# Autodesk Inventor assembly: mirrorHolder
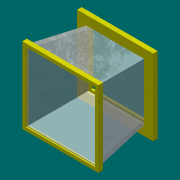
[picture p0: Inventor's stored thumbnail of the model, 180x180]
Saved by Autodesk Inventor 2016 (Build 200138000, 138)
## iProperties
Created: 2015-10-27
Part Number: mirrorHolder
Document SubType Name: Assembly
Designer: Sawaiz
Author: Sawaiz
## Documents named in this file (5)
- C:\Users\Sawaiz\OneDrive\projects\modularRICH\mirror\mirrorHolder.iam
- C:\Users\Sawaiz\OneDrive\projects\modularRICH\mirror\mirrorFrontFrame.ipt
- C:\Users\Sawaiz\OneDrive\projects\modularRICH\mirror\mirrorSides.ipt
- C:\Users\Sawaiz\OneDrive\projects\modularRICH\mirror\mirrorTopBottom.ipt
- C:\Users\Sawaiz\OneDrive\projects\modularRICH\mirror\mirrorBackFrame.ipt
## Components (6 placed, 4 different names)
1. mirrorFrontFrame:1 — Mate:7, Mate:8, Mate:9
2. mirrorSides:1 — Flush:2, Mate:5, Mate:6, Mate:9
3. mirrorTopBottom:1 — Flush:1, Mate:3, Mate:4, Mate:5, Mate:6
4. mirrorSides:2 — Flush:3, Mate:1, Mate:2, Mate:3, Mate:4
5. mirrorTopBottom:2 — Flush:1, Flush:2, Flush:3, Mate:1, Mate:2, Mate:7, Mate:8, Flush:4
6. mirrorBackFrame:1 — Flush:4
## Relationships (13: Mate 9, Flush 4)
- Flush:1: mirrorTopBottom:1 ↔ mirrorTopBottom:2
- Flush:2: mirrorSides:1 ↔ mirrorTopBottom:2
- Flush:3: mirrorSides:2 ↔ mirrorTopBottom:2
- Mate:1: mirrorSides:2 ↔ mirrorTopBottom:2
- Mate:2: mirrorSides:2 ↔ mirrorTopBottom:2
- Mate:3: mirrorTopBottom:1 ↔ mirrorSides:2
- Mate:4: mirrorTopBottom:1 ↔ mirrorSides:2
- Mate:5: mirrorSides:1 ↔ mirrorTopBottom:1
- Mate:6: mirrorSides:1 ↔ mirrorTopBottom:1
- Mate:7: mirrorFrontFrame:1 ↔ mirrorTopBottom:2
- Mate:8: mirrorFrontFrame:1 ↔ mirrorTopBottom:2
- Mate:9: mirrorFrontFrame:1 ↔ mirrorSides:1
- Flush:4: mirrorTopBottom:2 ↔ mirrorBackFrame:1
